# Autodesk Inventor assembly: Ankle
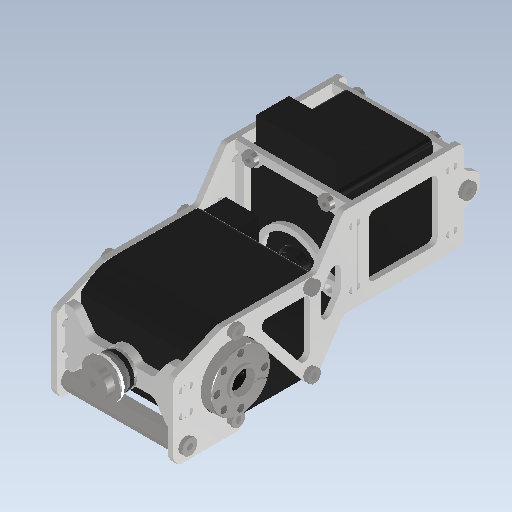
[picture p0: Inventor's stored thumbnail of the model, 512x512]
Saved by Autodesk Inventor 2020 (Build 240168000, 168)
## iProperties
Created: 2021-10-01
Part Number: Ankle
Document SubType Name: Assembly
Designer: Masato
Author: Masato
## Documents named in this file (21)
- C:\Users\MasatoKubotera\Documents\Inventor\OpenPlatform_ver3_0 - prototype\LowerBody\Ankle\Ankle.iam
- C:\Users\MasatoKubotera\Documents\Inventor\OpenPlatform_ver3_0 - prototype\ReadyMade\KONDO\B3M-SC-1040-A.ipt
- C:\Users\MasatoKubotera\Documents\Inventor\OpenPlatform_ver3_0 - prototype\ReadyMade\KONDO\B3M-SC-1170-A.ipt
- C:\Users\MasatoKubotera\Documents\Inventor\OpenPlatform_ver3_0 - prototype\ReadyMade\Spacer\SLSBF6-39.5-M3-N3.ipt
- C:\Users\MasatoKubotera\Documents\Inventor\OpenPlatform_ver3_0 - prototype\LowerBody\Ankle\Ankle_back_frame.ipt
- C:\Users\MasatoKubotera\Documents\Inventor\OpenPlatform_ver3_0 - prototype\LowerBody\Ankle\Ankle_front_frame.ipt
- C:\Users\MasatoKubotera\Documents\Inventor\OpenPlatform_ver3_0 - prototype\LowerBody\Ankle\Ankle_side_frame.ipt
- C:\Users\MasatoKubotera\Documents\Inventor\OpenPlatform_ver3_0 - prototype\ReadyMade\Screw\M2_6-15.ipt
- C:\Users\MasatoKubotera\Documents\Inventor\OpenPlatform_ver3_0 - prototype\ReadyMade\Screw\M2_6-20.ipt
- C:\Users\MasatoKubotera\Documents\Inventor\OpenPlatform_ver3_0 - prototype\ReadyMade\Screw\M3-6.ipt
- C:\Users\MasatoKubotera\Documents\Inventor\OpenPlatform_ver3_0 - prototype\ReadyMade\Bush\80F-0603.ipt
- C:\Users\MasatoKubotera\Documents\Inventor\OpenPlatform_ver3_0 - prototype\ReadyMade\KONDO\FreeHorn.ipt
- C:\Users\MasatoKubotera\Documents\Inventor\OpenPlatform_ver3_0 - prototype\ReadyMade\Washer\CC-0612-15B.ipt
- C:\Users\MasatoKubotera\Documents\Inventor\OpenPlatform_ver3_0 - prototype\ReadyMade\KONDO\FreeHorn_Screw.ipt
- C:\Users\MasatoKubotera\Documents\Inventor\OpenPlatform_ver3_0 - prototype\ReadyMade\InsertNut\S4-05-3W.ipt
- C:\Users\MasatoKubotera\Documents\Inventor\OpenPlatform_ver3_0 - prototype\ReadyMade\Washer\UUW-0412-10H.ipt
- C:\Users\MasatoKubotera\Documents\Inventor\OpenPlatform_ver3_0 - prototype\ReadyMade\Screw\DBTS4-6-4-DHC.ipt
- C:\Users\MasatoKubotera\Documents\Inventor\OpenPlatform_ver3_0 - prototype\ReadyMade\KONDO\ClampHorn.ipt
- C:\Users\MasatoKubotera\Documents\Inventor\OpenPlatform_ver3_0 - prototype\ReadyMade\Screw\620103008.ipt
- C:\Users\MasatoKubotera\Documents\Inventor\OpenPlatform_ver3_0 - prototype\ReadyMade\Washer\TT-0814-10.ipt
- C:\Users\MasatoKubotera\Documents\Inventor\OpenPlatform_ver3_0 - prototype\ReadyMade\Washer\UUW-0614-05H.ipt
## Components (40 placed, 20 different names)
1. B3M-SC-1170-A:1 — 挿入:1, 挿入:3, 挿入:4, 挿入:5, 挿入:7, 挿入:8, 挿入:42, 挿入:53, フラッシュ:4, フラッシュ:5, 挿入:60, 挿入:62, 角度:5
2. B3M-SC-1040-A:1 — 挿入:16, 挿入:17, 挿入:18, 挿入:43, 挿入:44, 挿入:58, 挿入:61, 挿入:63, 角度:6
3. SLSBF6-39.5-M3-N3:1 — 挿入:9, 挿入:10, 角度:2
4. SLSBF6-39.5-M3-N3:2 — 挿入:11, 挿入:12, 角度:3
5. Ankle_back_frame:1 — 挿入:16, 挿入:17, 挿入:18, メイト:7, メイト:6, フラッシュ:3, 挿入:37, 挿入:38, 挿入:39, 挿入:58, 挿入:59
6. Ankle_front_frame:1 — メイト:4, メイト:5, フラッシュ:1, 角度:4, 挿入:54, 挿入:55
7. Ankle_side_frame:1 — 挿入:5, 挿入:7, 挿入:8, 挿入:10, 挿入:12, メイト:4, メイト:5, フラッシュ:1, 挿入:23, 挿入:25, 挿入:26, 挿入:31, 挿入:32, メイト:7, メイト:6, フラッシュ:3, 角度:2, メイト:8, 挿入:64, 角度:3
8. Ankle_side_frame:2 — 挿入:1, 挿入:3, 挿入:4, 挿入:9, 挿入:11, 挿入:27, 挿入:28, 挿入:30, 挿入:33, 挿入:34, 挿入:65
9. 80F-0603:1 — 挿入:52
10. FreeHorn:1 — 挿入:42
11. Ankle_back_frame:2 — 挿入:43, 挿入:44, 挿入:47, 挿入:48
12. CC-0612-15B:1 — 挿入:52, 挿入:56
13. S4-05-3W:1 — 角度:4, 挿入:54
14. UUW-0412-10BH:1 — 挿入:55, 挿入:56, 挿入:57
15. DBS4-6-4:1 — 挿入:57, 挿入:66
16. ClampHorn:1 — 挿入:60, 角度:5
17. ClampHorn:2 — 挿入:61, 角度:6
18. TT-0814-10:1 — 挿入:67
19. UUW-0614-05BH:1 — 挿入:66, 挿入:67
20. 620103008:1 — 挿入:62
21. 620103008:2 — 挿入:63
22. FreeHorn_Screw:1 — 挿入:53
23. M3-6:1 — 挿入:31
24. M3-6:2 — 挿入:32
25. M3-6:3 — 挿入:33
26. M3-6:4 — 挿入:34
27. M2_6-15:1 — 挿入:26
28. M2_6-15:2 — 挿入:25
29. M2_6-15:3 — 挿入:64
30. M2_6-15:4 — 挿入:23
31. M2_6-15:5 — 挿入:37
32. M2_6-15:6 — 挿入:38
33. M2_6-15:7 — 挿入:39
34. M2_6-15:8 — 挿入:59
35. M2_6-20:1 — 挿入:27
36. M2_6-20:2 — 挿入:28
37. M2_6-20:3 — 挿入:65
38. M2_6-20:4 — 挿入:30
39. M2_6-20:5 — 挿入:47
40. M2_6-20:6 — 挿入:48
## Relationships (61: Insert 47, Mate 5, Angle 5, Flush 4)
- 挿入:1 [Insert]: B3M-SC-1170-A:1 ↔ Ankle_side_frame:2
- 挿入:3 [Insert]: B3M-SC-1170-A:1 ↔ Ankle_side_frame:2
- 挿入:4 [Insert]: B3M-SC-1170-A:1 ↔ Ankle_side_frame:2
- 挿入:5 [Insert]: B3M-SC-1170-A:1 ↔ Ankle_side_frame:1
- 挿入:7 [Insert]: B3M-SC-1170-A:1 ↔ Ankle_side_frame:1
- 挿入:8 [Insert]: B3M-SC-1170-A:1 ↔ Ankle_side_frame:1
- 挿入:9 [Insert]: SLSBF6-39.5-M3-N3:1 ↔ Ankle_side_frame:2
- 挿入:10 [Insert]: SLSBF6-39.5-M3-N3:1 ↔ Ankle_side_frame:1
- 挿入:11 [Insert]: SLSBF6-39.5-M3-N3:2 ↔ Ankle_side_frame:2
- 挿入:12 [Insert]: SLSBF6-39.5-M3-N3:2 ↔ Ankle_side_frame:1
- 挿入:16 [Insert]: B3M-SC-1040-A:1 ↔ Ankle_back_frame:1
- 挿入:17 [Insert]: B3M-SC-1040-A:1 ↔ Ankle_back_frame:1
- 挿入:18 [Insert]: B3M-SC-1040-A:1 ↔ Ankle_back_frame:1
- メイト:4 [Mate] (0.025 mm): Ankle_front_frame:1 ↔ Ankle_side_frame:1
- メイト:5 [Mate] (0.025 mm): Ankle_front_frame:1 ↔ Ankle_side_frame:1
- フラッシュ:1 [Flush]: Ankle_front_frame:1 ↔ Ankle_side_frame:1
- 角度:2 [Angle] (0 deg): SLSBF6-39.5-M3-N3:1 ↔ Ankle_side_frame:1
- 挿入:23 [Insert]: Ankle_side_frame:1 ↔ M2_6-15:4
- 挿入:25 [Insert]: Ankle_side_frame:1 ↔ M2_6-15:2
- 挿入:26 [Insert]: Ankle_side_frame:1 ↔ M2_6-15:1
- 挿入:27 [Insert]: Ankle_side_frame:2 ↔ M2_6-20:1
- 挿入:28 [Insert]: Ankle_side_frame:2 ↔ M2_6-20:2
- 挿入:30 [Insert]: Ankle_side_frame:2 ↔ M2_6-20:4
- 挿入:31 [Insert]: Ankle_side_frame:1 ↔ M3-6:1
- 挿入:32 [Insert]: Ankle_side_frame:1 ↔ M3-6:2
- 挿入:33 [Insert]: Ankle_side_frame:2 ↔ M3-6:3
- 挿入:34 [Insert]: Ankle_side_frame:2 ↔ M3-6:4
- メイト:7 [Mate] (0.025 mm): Ankle_back_frame:1 ↔ Ankle_side_frame:1
- メイト:6 [Mate] (0.025 mm): Ankle_back_frame:1 ↔ Ankle_side_frame:1
- フラッシュ:3 [Flush]: Ankle_back_frame:1 ↔ Ankle_side_frame:1
- 挿入:37 [Insert]: Ankle_back_frame:1 ↔ M2_6-15:5
- 挿入:38 [Insert]: Ankle_back_frame:1 ↔ M2_6-15:6
- 挿入:39 [Insert]: Ankle_back_frame:1 ↔ M2_6-15:7
- 角度:3 [Angle] (0 deg): SLSBF6-39.5-M3-N3:2 ↔ Ankle_side_frame:1
- 挿入:42 [Insert]: B3M-SC-1170-A:1 ↔ FreeHorn:1
- 挿入:43 [Insert]: B3M-SC-1040-A:1 ↔ Ankle_back_frame:2
- 挿入:44 [Insert]: B3M-SC-1040-A:1 ↔ Ankle_back_frame:2
- 挿入:47 [Insert]: Ankle_back_frame:2 ↔ M2_6-20:5
- 挿入:48 [Insert]: Ankle_back_frame:2 ↔ M2_6-20:6
- 挿入:52 [Insert]: 80F-0603:1 ↔ CC-0612-15B:1
- 挿入:53 [Insert]: B3M-SC-1170-A:1 ↔ FreeHorn_Screw:1
- 角度:4 [Angle] (0 deg): Ankle_front_frame:1 ↔ S4-05-3W:1
- 挿入:54 [Insert]: Ankle_front_frame:1 ↔ S4-05-3W:1
- 挿入:55 [Insert]: Ankle_front_frame:1 ↔ UUW-0412-10BH:1
- 挿入:56 [Insert]: CC-0612-15B:1 ↔ UUW-0412-10BH:1
- 挿入:57 [Insert]: UUW-0412-10BH:1 ↔ DBS4-6-4:1
- 挿入:58 [Insert]: B3M-SC-1040-A:1 ↔ Ankle_back_frame:1
- 挿入:59 [Insert]: Ankle_back_frame:1 ↔ M2_6-15:8
- メイト:8 [Mate] (19.75 mm): Ankle_side_frame:1
- フラッシュ:4 [Flush]: B3M-SC-1170-A:1
- フラッシュ:5 [Flush]: B3M-SC-1170-A:1
- 挿入:60 [Insert]: B3M-SC-1170-A:1 ↔ ClampHorn:1
- 挿入:61 [Insert]: B3M-SC-1040-A:1 ↔ ClampHorn:2
- 挿入:62 [Insert]: B3M-SC-1170-A:1 ↔ 620103008:1
- 挿入:63 [Insert]: B3M-SC-1040-A:1 ↔ 620103008:2
- 角度:5 [Angle] (0 deg): B3M-SC-1170-A:1 ↔ ClampHorn:1
- 角度:6 [Angle] (0 deg): B3M-SC-1040-A:1 ↔ ClampHorn:2
- 挿入:64 [Insert]: Ankle_side_frame:1 ↔ M2_6-15:3
- 挿入:65 [Insert]: Ankle_side_frame:2 ↔ M2_6-20:3
- 挿入:66 [Insert]: DBS4-6-4:1 ↔ UUW-0614-05BH:1
- 挿入:67 [Insert]: TT-0814-10:1 ↔ UUW-0614-05BH:1
